# Autodesk Inventor assembly: PCB_board_box
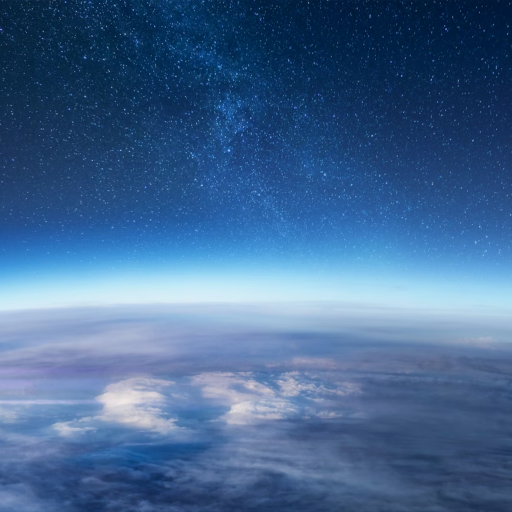
[picture p0: Inventor's stored thumbnail of the model, 512x512]
Saved by Autodesk Inventor 2023 (Build 270158000, 158)
## iProperties
Created: 2023-05-25
Part Number: PCB_board_box
Document SubType Name: Assembly
Designer: 310611102
Author: 310611102
## Documents named in this file (10)
- C:\Users\310611102\Documents\Inventor\SSR\avionics_2023ver\electronics\shield box\shieldbox_ver2\PCB_board_box.iam
- C:\Users\310611102\Documents\Inventor\SSR\avionics_2023ver\electronics\shield box\shieldbox_ver2\PCB_board_box_buttom.ipt
- C:\Users\310611102\Documents\Inventor\SSR\avionics_2023ver\electronics\shield box\shieldbox_ver2\PCB_board_box_front.ipt
- C:\Users\310611102\Documents\Inventor\SSR\avionics_2023ver\electronics\shield box\shieldbox_ver2\PCB_board_box_left.ipt
- C:\Users\310611102\Documents\Inventor\SSR\avionics_2023ver\electronics\shield box\shieldbox_ver2\PCB_board_box_right.ipt
- C:\Users\310611102\Documents\Inventor\SSR\avionics_2023ver\electronics\shield box\shieldbox_ver2\PCB_board_box_top.ipt
- C:\Users\310611102\Documents\Inventor\SSR\avionics_2023ver\electronics\shield box\shieldbox_ver2\PCB_board_box_back.ipt
- C:\Users\310611102\Documents\Inventor\SSR\avionics_2023ver\electronics\shield box\shieldbox_ver2\connector.ipt
- C:\Users\310611102\Documents\Inventor\SSR\avionics_2023ver\electronics\ISO 10642 - M3 x  8.ipt
- C:\Users\310611102\Documents\Inventor\SSR\avionics_2023ver\electronics\ISO 4032 - M3 - ISO.ipt
## Components (74 placed, 9 different names)
1. PCB_board_box_buttom:1 — Insert:26, Insert:28, Mate:7, Cylindrical:3, Cylindrical:4, Cylindrical:7, Cylindrical:8, Cylindrical:19, Angle:1, Mate:9, Insert:52, Insert:53, Insert:57, Insert:58, Insert:59, Insert:60
2. PCB_board_box_front:1 — Mate:3, Insert:30, Mate:8, Cylindrical:5, Cylindrical:9, Cylindrical:10, Cylindrical:11, Insert:38, Insert:61, Insert:62, Insert:63, Insert:64, Insert:66, Insert:67
3. PCB_board_box_left:1 — Insert:22, Insert:23, Insert:25, Mate:2, Mate:3, Insert:31
4. PCB_board_box_right:1 — Insert:35, Insert:37, Insert:40, Insert:41, Insert:42, Insert:44
5. PCB_board_box_top:1 — Mate:8, Cylindrical:12, Cylindrical:13, Insert:34, Cylindrical:15, Cylindrical:17, Insert:47, Insert:68, Insert:69, Insert:70, Insert:71
6. PCB_board_box_back:1 — Insert:24, Mate:2, Mate:7, Cylindrical:6, Cylindrical:14, Cylindrical:16, Cylindrical:18, Insert:39, Angle:2, Insert:43, Insert:45, Insert:46, Insert:48, Insert:49, Insert:50
7. ISO 10642 M3x8:1 — Insert:41
8. ISO 10642 M3x8:2 — Insert:42
9. ISO 10642 M3x8:3 — Insert:43
10. ISO 10642 M3x8:4 — Insert:44
11. ISO 10642 M3x8:5 — Insert:45
12. ISO 10642 M3x8:6 — Insert:46
13. ISO 10642 M3x8:7 — Insert:47
14. ISO 10642 M3x8:8 — Insert:48
15. ISO 10642 M3x8:9 — Insert:49
16. ISO 10642 M3x8:10 — Insert:50
17. ISO 10642 M3x8:12 — Insert:52
18. ISO 10642 M3x8:13 — Insert:53
19. ISO 10642 M3x8:16 — Insert:57
20. ISO 10642 M3x8:17 — Insert:58
21. ISO 10642 M3x8:18 — Insert:59
22. ISO 10642 M3x8:19 — Insert:60
23. ISO 10642 M3x8:20 — Insert:61
24. ISO 10642 M3x8:21 — Insert:62
25. ISO 10642 M3x8:22 — Insert:63
26. ISO 10642 M3x8:23 — Insert:64
27. ISO 10642 M3x8:25 — Insert:66
28. ISO 10642 M3x8:26 — Insert:67
29. ISO 10642 M3x8:27 — Insert:68
30. ISO 10642 M3x8:28 — Insert:69
31. ISO 10642 M3x8:29 — Insert:70
32. ISO 10642 M3x8:30 — Insert:71
33. ISO 4032 M3:1 — Insert:72
34. ISO 4032 M3:2 — Insert:73
35. ISO 4032 M3:3 — Insert:74
36. ISO 4032 M3:4 — Insert:75
37. ISO 4032 M3:5 — Insert:76
38. ISO 4032 M3:6 — Insert:77
39. ISO 4032 M3:7 — Insert:78
40. ISO 4032 M3:8 — Insert:79
41. ISO 4032 M3:9 — Insert:80
42. ISO 4032 M3:10 — Insert:81
43. ISO 4032 M3:11 — Insert:82
44. ISO 4032 M3:12 — Insert:83
45. ISO 4032 M3:13 — Insert:84
46. ISO 4032 M3:14 — Insert:85
47. ISO 4032 M3:15 — Insert:86
48. ISO 4032 M3:16 — Insert:87
49. ISO 4032 M3:17 — Insert:88
50. ISO 4032 M3:18 — Insert:89
51. ISO 4032 M3:19 — Insert:90
52. ISO 4032 M3:20 — Insert:91
53. ISO 4032 M3:21 — Insert:92
54. ISO 4032 M3:22 — Insert:93
55. ISO 4032 M3:23 — Insert:94
56. ISO 4032 M3:24 — Insert:95
57. ISO 4032 M3:25 — Insert:96
58. ISO 4032 M3:26 — Insert:97
59. connector:1 — Insert:37, Insert:38, Insert:96, Insert:97
60. connector:2 — Cylindrical:4, Cylindrical:5, Insert:92, Insert:94
61. connector:4 — Cylindrical:14, Cylindrical:15, Insert:77, Insert:82
62. connector:6 — Insert:23, Insert:26, Insert:90
63. connector:7 — Insert:24, Insert:25, Insert:83
64. connector:8 — Insert:22, Insert:28, Insert:91
65. connector:10 — Insert:30, Insert:31, Insert:76
66. connector:11 — Cylindrical:3, Cylindrical:6, Insert:88, Insert:89
67. connector:12 — Cylindrical:16, Cylindrical:17, Insert:78, Insert:81
68. connector:13 — Cylindrical:7
69. connector:14 — Cylindrical:8, Cylindrical:9, Insert:93, Insert:95
70. connector:15 — Cylindrical:10, Cylindrical:12, Insert:72, Insert:73
71. connector:16 — Cylindrical:11, Cylindrical:13, Insert:74, Insert:75
72. connector:17 — Insert:34, Insert:35, Insert:79, Insert:80
73. connector:18 — Cylindrical:18, Cylindrical:19, Insert:86, Insert:87
74. connector:19 — Insert:39, Insert:40, Insert:84, Insert:85
## Relationships (90: Insert 66, CylindricalJoint 17, Mate 5, Angle 2)
- Insert:22: PCB_board_box_left:1 ↔ connector:8
- Insert:23: PCB_board_box_left:1 ↔ connector:6
- Insert:24: PCB_board_box_back:1 ↔ connector:7
- Insert:25: PCB_board_box_left:1 ↔ connector:7
- Mate:2: PCB_board_box_left:1 ↔ PCB_board_box_back:1
- Insert:26: PCB_board_box_buttom:1 ↔ connector:6
- Mate:3: PCB_board_box_front:1 ↔ PCB_board_box_left:1
- Insert:28: PCB_board_box_buttom:1 ↔ connector:8
- Mate:7: PCB_board_box_buttom:1 ↔ PCB_board_box_back:1
- Cylindrical:3: PCB_board_box_buttom:1 ↔ connector:11
- Insert:30: PCB_board_box_front:1 ↔ connector:10
- Insert:31: PCB_board_box_left:1 ↔ connector:10
- Mate:8: PCB_board_box_front:1 ↔ PCB_board_box_top:1
- Cylindrical:4: PCB_board_box_buttom:1 ↔ connector:2
- Cylindrical:5: PCB_board_box_front:1 ↔ connector:2
- Cylindrical:6: PCB_board_box_back:1 ↔ connector:11
- Cylindrical:7: PCB_board_box_buttom:1 ↔ connector:13
- Cylindrical:8: PCB_board_box_buttom:1 ↔ connector:14
- Cylindrical:9: PCB_board_box_front:1 ↔ connector:14
- Cylindrical:10: PCB_board_box_front:1 ↔ connector:15
- Cylindrical:11: PCB_board_box_front:1 ↔ connector:16
- Cylindrical:12: PCB_board_box_top:1 ↔ connector:15
- Cylindrical:13: PCB_board_box_top:1 ↔ connector:16
- Insert:34: PCB_board_box_top:1 ↔ connector:17
- Cylindrical:14: PCB_board_box_back:1 ↔ connector:4
- Cylindrical:15: PCB_board_box_top:1 ↔ connector:4
- Cylindrical:16: PCB_board_box_back:1 ↔ connector:12
- Cylindrical:17: PCB_board_box_top:1 ↔ connector:12
- Insert:35: PCB_board_box_right:1 ↔ connector:17
- Cylindrical:18: PCB_board_box_back:1 ↔ connector:18
- Cylindrical:19: PCB_board_box_buttom:1 ↔ connector:18
- Insert:37: PCB_board_box_right:1 ↔ connector:1
- Insert:38: PCB_board_box_front:1 ↔ connector:1
- Insert:39: PCB_board_box_back:1 ↔ connector:19
- Insert:40: PCB_board_box_right:1 ↔ connector:19
- Angle:1 (0 deg): PCB_board_box_buttom:1
- Angle:2 (180 deg): PCB_board_box_back:1
- Mate:9: PCB_board_box_buttom:1
- Insert:41: PCB_board_box_right:1 ↔ ISO 10642 M3x8:1
- Insert:42: PCB_board_box_right:1 ↔ ISO 10642 M3x8:2
- Insert:43: PCB_board_box_back:1 ↔ ISO 10642 M3x8:3
- Insert:44: PCB_board_box_right:1 ↔ ISO 10642 M3x8:4
- Insert:45: PCB_board_box_back:1 ↔ ISO 10642 M3x8:5
- Insert:46: PCB_board_box_back:1 ↔ ISO 10642 M3x8:6
- Insert:47: PCB_board_box_top:1 ↔ ISO 10642 M3x8:7
- Insert:48: PCB_board_box_back:1 ↔ ISO 10642 M3x8:8
- Insert:49: PCB_board_box_back:1 ↔ ISO 10642 M3x8:9
- Insert:50: PCB_board_box_back:1 ↔ ISO 10642 M3x8:10
- Insert:52: PCB_board_box_buttom:1 ↔ ISO 10642 M3x8:12
- Insert:53: PCB_board_box_buttom:1 ↔ ISO 10642 M3x8:13
- Insert:57: PCB_board_box_buttom:1 ↔ ISO 10642 M3x8:16
- Insert:58: PCB_board_box_buttom:1 ↔ ISO 10642 M3x8:17
- Insert:59: PCB_board_box_buttom:1 ↔ ISO 10642 M3x8:18
- Insert:60: PCB_board_box_buttom:1 ↔ ISO 10642 M3x8:19
- Insert:61: PCB_board_box_front:1 ↔ ISO 10642 M3x8:20
- Insert:62: PCB_board_box_front:1 ↔ ISO 10642 M3x8:21
- Insert:63: PCB_board_box_front:1 ↔ ISO 10642 M3x8:22
- Insert:64: PCB_board_box_front:1 ↔ ISO 10642 M3x8:23
- Insert:66: PCB_board_box_front:1 ↔ ISO 10642 M3x8:25
- Insert:67: PCB_board_box_front:1 ↔ ISO 10642 M3x8:26
- Insert:68: PCB_board_box_top:1 ↔ ISO 10642 M3x8:27
- Insert:69: PCB_board_box_top:1 ↔ ISO 10642 M3x8:28
- Insert:70: PCB_board_box_top:1 ↔ ISO 10642 M3x8:29
- Insert:71: PCB_board_box_top:1 ↔ ISO 10642 M3x8:30
- Insert:72: ISO 4032 M3:1 ↔ connector:15
- Insert:73: ISO 4032 M3:2 ↔ connector:15
- Insert:74: ISO 4032 M3:3 ↔ connector:16
- Insert:75: ISO 4032 M3:4 ↔ connector:16
- Insert:76: ISO 4032 M3:5 ↔ connector:10
- Insert:77: ISO 4032 M3:6 ↔ connector:4
- Insert:78: ISO 4032 M3:7 ↔ connector:12
- Insert:79: ISO 4032 M3:8 ↔ connector:17
- Insert:80: ISO 4032 M3:9 ↔ connector:17
- Insert:81: ISO 4032 M3:10 ↔ connector:12
- Insert:82: ISO 4032 M3:11 ↔ connector:4
- Insert:83: ISO 4032 M3:12 ↔ connector:7
- Insert:84: ISO 4032 M3:13 ↔ connector:19
- Insert:85: ISO 4032 M3:14 ↔ connector:19
- Insert:86: ISO 4032 M3:15 ↔ connector:18
- Insert:87: ISO 4032 M3:16 ↔ connector:18
- Insert:88: ISO 4032 M3:17 ↔ connector:11
- Insert:89: ISO 4032 M3:18 ↔ connector:11
- Insert:90: ISO 4032 M3:19 ↔ connector:6
- Insert:91: ISO 4032 M3:20 ↔ connector:8
- Insert:92: ISO 4032 M3:21 ↔ connector:2
- Insert:93: ISO 4032 M3:22 ↔ connector:14
- Insert:94: ISO 4032 M3:23 ↔ connector:2
- Insert:95: ISO 4032 M3:24 ↔ connector:14
- Insert:96: ISO 4032 M3:25 ↔ connector:1
- Insert:97: ISO 4032 M3:26 ↔ connector:1
